# Autodesk Inventor assembly: prog to kauri rear link mod
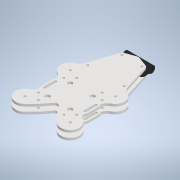
[picture p0: Inventor's stored thumbnail of the model, 180x180]
Saved by Autodesk Inventor 2020 (Build 240168000, 168)
## iProperties
Created: 2022-05-24
Part Number: prog to kauri rear link mod
Document SubType Name: Assembly
Designer: Steven
Author: Steven
## Documents named in this file (3)
- Y:\FPV drone stuff\0 Street League\Frames\experimental-quad-frames\prog to kauri rear link mod.iam
- Y:\FPV drone stuff\0 Street League\Frames\experimental-quad-frames\399 prig z plate.ipt
- Y:\FPV drone stuff\0 Street League\Frames\PB-Kauri-X\3D prints\35 mm canopy\KauriRearLink 35mm no brass insert.ipt
## Components (3 placed, 2 different names)
1. 399 prig z plate:1 — Mate:1, Mate:2, Mate:3, Mate:5
2. 399 prig z plate:2 — Mate:1, Mate:2, Mate:3, Mate:4, Mate:6
3. KauriRearLink 35mm no brass insert:1 — Mate:4, Mate:5, Mate:6
## Relationships (6: Mate 6)
- Mate:1 (6 mm): 399 prig z plate:1 ↔ 399 prig z plate:2
- Mate:2: 399 prig z plate:1 ↔ 399 prig z plate:2
- Mate:3: 399 prig z plate:1 ↔ 399 prig z plate:2
- Mate:4: 399 prig z plate:2 ↔ KauriRearLink 35mm no brass insert:1
- Mate:5: 399 prig z plate:1 ↔ KauriRearLink 35mm no brass insert:1
- Mate:6: 399 prig z plate:2 ↔ KauriRearLink 35mm no brass insert:1
